# Autodesk Inventor assembly: Gehäuse
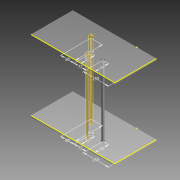
[picture p0: Inventor's stored thumbnail of the model, 180x180]
Saved by Autodesk Inventor 2013 (Build 170138000, 138)
## iProperties
Created: 2012-10-19
Part Number: Gehäuse
Document SubType Name: Assembly
Designer: fivef
Author: fivef
## Documents named in this file (5)
- D:\Dropbox\My Dropbox\Dokumente\Aktuell\Drinkmixer\Gehäuse.iam
- D:\Dropbox\My Dropbox\Dokumente\Aktuell\Drinkmixer\Zwischenstange.ipt
- D:\Dropbox\My Dropbox\Dokumente\Aktuell\Drinkmixer\Wand rechts.ipt
- D:\Dropbox\My Dropbox\Dokumente\Aktuell\Drinkmixer\Zwischenstange_CPY.ipt
- D:\Dropbox\My Dropbox\Dokumente\Aktuell\Drinkmixer\zwischenstab.iam
## Components (5 placed, 5 different names)
1. seitenwand rechts:1 — Passend:1, Passend:8, Passend:13, Fluchtend:3, Passend:14, Passend:15
2. seitenwand kopie (links):2 — Passend:5, Passend:7, Fluchtend:3
3. zwischenstab:1 [sub-assembly] — Passend:14, Passend:15
4. Zwischenstange:1 — Passend:1, Passend:5
5. Zwischenstange_schlauchhalter:1 — Passend:7, Passend:8, Passend:13
## Relationships (8: Mate 7, Flush 1)
- Passend:1 [Mate]: seitenwand rechts:1 ↔ Zwischenstange:1
- Passend:5 [Mate]: seitenwand kopie (links):2 ↔ Zwischenstange:1
- Passend:7 [Mate]: seitenwand kopie (links):2 ↔ Zwischenstange_schlauchhalter:1
- Passend:8 [Mate]: seitenwand rechts:1 ↔ Zwischenstange_schlauchhalter:1
- Passend:13 [Mate]: seitenwand rechts:1 ↔ Zwischenstange_schlauchhalter:1
- Fluchtend:3 [Flush]: seitenwand rechts:1 ↔ seitenwand kopie (links):2
- Passend:14 [Mate]: seitenwand rechts:1 ↔ zwischenstab:1
- Passend:15 [Mate]: seitenwand rechts:1 ↔ zwischenstab:1
